# Autodesk Inventor assembly: leg_Left_femur_ass
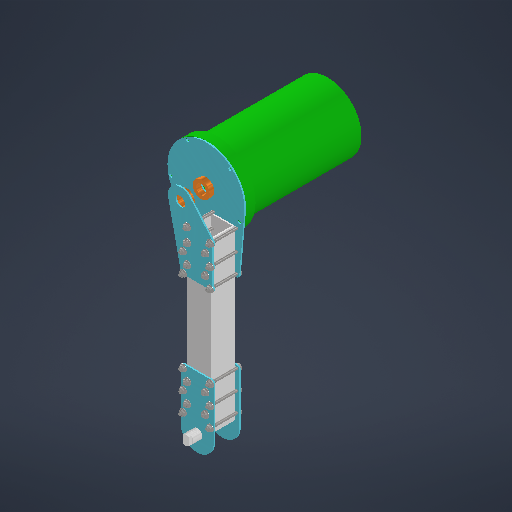
[picture p0: Inventor's stored thumbnail of the model, 512x512]
Saved by Autodesk Inventor 2026 (Build 300175000, 175)
## iProperties
Created: 2026-04-24
Part Number: leg_Left_femur_ass
Document SubType Name: Assembly
Designer: user
Mass: 5132.93 g
Surface Area: 5038.46 cm^2
Volume: 3187.52 cm^3
Density: 1.61032 g/cm^3
Author: user
## Documents named in this file (11)
- C:\Users\user\Documents\spider_metal\leg_femur\leg_Left_femur_ass.iam
- C:\Users\user\Documents\spider_metal\leg_femur\femur_profile.ipt
- C:\Users\user\Documents\spider_metal\leg_femur\femur_support_steel.ipt
- C:\Users\user\Documents\spider_metal\leg_femur\femur_motor_steel.ipt
- C:\Users\user\Documents\spider_metal\leg_femur\femur_outside_steel.ipt
- C:\Users\user\Documents\Inventor\Content Center Files\R2026\ru-RU\GOST 7805-70\Болт M6-6gx65 ГОСТ 7805-70.ipt
- C:\Users\user\Documents\Inventor\Content Center Files\R2026\ru-RU\Nut GOST R 50592-93\Гайка M6-6H ГОСТ Р 50592-93.ipt
- C:\Users\user\Documents\Inventor\Content Center Files\R2026\ru-RU\GOST 7798-70\Болт M6-6gx65 ГОСТ 7798-70.ipt
- C:\Users\user\Documents\spider_metal\leg_femur\shaft_femur.ipt
- C:\Users\user\Documents\spider_metal\body_parts\motor_mass.ipt
- C:\Users\user\Documents\spider_metal\body_parts\bearing_mass.ipt
## Components (49 placed, 10 different names)
1. femur_profile:1 — Жесткий:1, Жесткий:2, Жесткий:3, Жесткий:4, Совмещение:47, Совмещение:67
2. femur_support_steel:1 — Жесткий:1, Совмещение:22, Совмещение:24, Совмещение:26, Совмещение:28, Совмещение:30, Совмещение:32, Совмещение:34, Совмещение:36, Совмещение:38, Совмещение:40, С поворотом:3
3. femur_motor_steel:1 — Жесткий:4, Совмещение:1, Совмещение:2, Совмещение:3, Совмещение:4, Совмещение:5, Совмещение:6, Совмещение:7, Совмещение:8, Совмещение:9, Совмещение:10, Совмещение:11, Совмещение:12, Совмещение:13, Совмещение:14, Совмещение:15, Совмещение:16, Совмещение:17, Совмещение:18, Совмещение:19, Совмещение:20, Совмещение:21, Совмещение:23, Совмещение:25, Совмещение:27, Совмещение:29, Совмещение:31, Совмещение:33, Совмещение:35, Совмещение:37, Совмещение:39, С поворотом:1, Жесткий:6, С поворотом:2
4. femur_outside_steel:1 — Жесткий:2, Совмещение:62, Совмещение:64, Совмещение:66, Совмещение:68, Совмещение:70, Совмещение:72, Совмещение:74, Совмещение:76, Совмещение:78, Совмещение:80
5. femur_outside_steel:2 — Жесткий:3, Совмещение:41, Совмещение:42, Совмещение:43, Совмещение:44, Совмещение:45, Совмещение:46, Совмещение:48, Совмещение:49, Совмещение:50, Совмещение:51, Совмещение:52, Совмещение:53, Совмещение:54, Совмещение:55, Совмещение:56, Совмещение:57, Совмещение:58, Совмещение:59, Совмещение:60, Совмещение:61, Совмещение:63, Совмещение:65, Совмещение:69, Совмещение:71, Совмещение:73, Совмещение:75, Совмещение:77, Совмещение:79, Жесткий:5
6. shaft_femur:1 — Жесткий:5
7. motor_mass:1 — С поворотом:1, Жесткий:6
8. bearing_mass:1 — С поворотом:2
9. bearing_mass:2 — С поворотом:3
10. Болт ГОСТ 7798-70 - Отозвано M6-6gx65:1 — Совмещение:41, Совмещение:42
11. Гайка ГОСТ Р 50592-93 M6:11 — Совмещение:61, Совмещение:62
12. Болт ГОСТ 7798-70 - Отозвано M6-6gx65:2 — Совмещение:43, Совмещение:44
13. Болт ГОСТ 7798-70 - Отозвано M6-6gx65:3 — Совмещение:45, Совмещение:46
14. Болт ГОСТ 7798-70 - Отозвано M6-6gx65:4 — Совмещение:47, Совмещение:48
15. Болт ГОСТ 7798-70 - Отозвано M6-6gx65:5 — Совмещение:49, Совмещение:50
16. Болт ГОСТ 7798-70 - Отозвано M6-6gx65:6 — Совмещение:51, Совмещение:52
17. Болт ГОСТ 7798-70 - Отозвано M6-6gx65:7 — Совмещение:53, Совмещение:54
18. Болт ГОСТ 7798-70 - Отозвано M6-6gx65:8 — Совмещение:55, Совмещение:56
19. Болт ГОСТ 7798-70 - Отозвано M6-6gx65:9 — Совмещение:57, Совмещение:58
20. Болт ГОСТ 7798-70 - Отозвано M6-6gx65:10 — Совмещение:59, Совмещение:60
21. Гайка ГОСТ Р 50592-93 M6:12 — Совмещение:63, Совмещение:64
22. Гайка ГОСТ Р 50592-93 M6:13 — Совмещение:65, Совмещение:66
23. Гайка ГОСТ Р 50592-93 M6:14 — Совмещение:67, Совмещение:68
24. Гайка ГОСТ Р 50592-93 M6:15 — Совмещение:69, Совмещение:70
25. Гайка ГОСТ Р 50592-93 M6:16 — Совмещение:71, Совмещение:72
26. Гайка ГОСТ Р 50592-93 M6:17 — Совмещение:73, Совмещение:74
27. Гайка ГОСТ Р 50592-93 M6:18 — Совмещение:75, Совмещение:76
28. Гайка ГОСТ Р 50592-93 M6:19 — Совмещение:77, Совмещение:78
29. Гайка ГОСТ Р 50592-93 M6:20 — Совмещение:79, Совмещение:80
30. Болт ГОСТ 7805-70 M6-6gx65:1 — Совмещение:1, Совмещение:2
31. Гайка ГОСТ Р 50592-93 M6:1 — Совмещение:21, Совмещение:22
32. Болт ГОСТ 7805-70 M6-6gx65:2 — Совмещение:3, Совмещение:4
33. Болт ГОСТ 7805-70 M6-6gx65:3 — Совмещение:5, Совмещение:6
34. Болт ГОСТ 7805-70 M6-6gx65:4 — Совмещение:7, Совмещение:8
35. Болт ГОСТ 7805-70 M6-6gx65:5 — Совмещение:9, Совмещение:10
36. Болт ГОСТ 7805-70 M6-6gx65:6 — Совмещение:11, Совмещение:12
37. Болт ГОСТ 7805-70 M6-6gx65:7 — Совмещение:13, Совмещение:14
38. Болт ГОСТ 7805-70 M6-6gx65:8 — Совмещение:15, Совмещение:16
39. Болт ГОСТ 7805-70 M6-6gx65:9 — Совмещение:17, Совмещение:18
40. Болт ГОСТ 7805-70 M6-6gx65:10 — Совмещение:19, Совмещение:20
41. Гайка ГОСТ Р 50592-93 M6:2 — Совмещение:23, Совмещение:24
42. Гайка ГОСТ Р 50592-93 M6:3 — Совмещение:25, Совмещение:26
43. Гайка ГОСТ Р 50592-93 M6:4 — Совмещение:27, Совмещение:28
44. Гайка ГОСТ Р 50592-93 M6:5 — Совмещение:29, Совмещение:30
45. Гайка ГОСТ Р 50592-93 M6:6 — Совмещение:31, Совмещение:32
46. Гайка ГОСТ Р 50592-93 M6:7 — Совмещение:33, Совмещение:34
47. Гайка ГОСТ Р 50592-93 M6:8 — Совмещение:35, Совмещение:36
48. Гайка ГОСТ Р 50592-93 M6:9 — Совмещение:37, Совмещение:38
49. Гайка ГОСТ Р 50592-93 M6:10 — Совмещение:39, Совмещение:40
## Relationships (89: Mate 80, WeldJoint 6, RevoluteJoint 3)
- Жесткий:1 [WeldJoint]: femur_profile:1 ↔ femur_support_steel:1
- Жесткий:2 [WeldJoint]: femur_profile:1 ↔ femur_outside_steel:1
- Жесткий:3 [WeldJoint]: femur_profile:1 ↔ femur_outside_steel:2
- Жесткий:4 [WeldJoint]: femur_profile:1 ↔ femur_motor_steel:1
- Совмещение:1 [Mate]: femur_motor_steel:1 ↔ Болт ГОСТ 7805-70 M6-6gx65:1
- Совмещение:2 [Mate]: femur_motor_steel:1 ↔ Болт ГОСТ 7805-70 M6-6gx65:1
- Совмещение:3 [Mate]: femur_motor_steel:1 ↔ Болт ГОСТ 7805-70 M6-6gx65:2
- Совмещение:4 [Mate]: femur_motor_steel:1 ↔ Болт ГОСТ 7805-70 M6-6gx65:2
- Совмещение:5 [Mate]: femur_motor_steel:1 ↔ Болт ГОСТ 7805-70 M6-6gx65:3
- Совмещение:6 [Mate]: femur_motor_steel:1 ↔ Болт ГОСТ 7805-70 M6-6gx65:3
- Совмещение:7 [Mate]: femur_motor_steel:1 ↔ Болт ГОСТ 7805-70 M6-6gx65:4
- Совмещение:8 [Mate]: femur_motor_steel:1 ↔ Болт ГОСТ 7805-70 M6-6gx65:4
- Совмещение:9 [Mate]: femur_motor_steel:1 ↔ Болт ГОСТ 7805-70 M6-6gx65:5
- Совмещение:10 [Mate]: femur_motor_steel:1 ↔ Болт ГОСТ 7805-70 M6-6gx65:5
- Совмещение:11 [Mate]: femur_motor_steel:1 ↔ Болт ГОСТ 7805-70 M6-6gx65:6
- Совмещение:12 [Mate]: femur_motor_steel:1 ↔ Болт ГОСТ 7805-70 M6-6gx65:6
- Совмещение:13 [Mate]: femur_motor_steel:1 ↔ Болт ГОСТ 7805-70 M6-6gx65:7
- Совмещение:14 [Mate]: femur_motor_steel:1 ↔ Болт ГОСТ 7805-70 M6-6gx65:7
- Совмещение:15 [Mate]: femur_motor_steel:1 ↔ Болт ГОСТ 7805-70 M6-6gx65:8
- Совмещение:16 [Mate]: femur_motor_steel:1 ↔ Болт ГОСТ 7805-70 M6-6gx65:8
- Совмещение:17 [Mate]: femur_motor_steel:1 ↔ Болт ГОСТ 7805-70 M6-6gx65:9
- Совмещение:18 [Mate]: femur_motor_steel:1 ↔ Болт ГОСТ 7805-70 M6-6gx65:9
- Совмещение:19 [Mate]: femur_motor_steel:1 ↔ Болт ГОСТ 7805-70 M6-6gx65:10
- Совмещение:20 [Mate]: femur_motor_steel:1 ↔ Болт ГОСТ 7805-70 M6-6gx65:10
- Совмещение:21 [Mate]: femur_motor_steel:1 ↔ Гайка ГОСТ Р 50592-93 M6:1
- Совмещение:22 [Mate]: femur_support_steel:1 ↔ Гайка ГОСТ Р 50592-93 M6:1
- Совмещение:23 [Mate]: femur_motor_steel:1 ↔ Гайка ГОСТ Р 50592-93 M6:2
- Совмещение:24 [Mate]: femur_support_steel:1 ↔ Гайка ГОСТ Р 50592-93 M6:2
- Совмещение:25 [Mate]: femur_motor_steel:1 ↔ Гайка ГОСТ Р 50592-93 M6:3
- Совмещение:26 [Mate]: femur_support_steel:1 ↔ Гайка ГОСТ Р 50592-93 M6:3
- Совмещение:27 [Mate]: femur_motor_steel:1 ↔ Гайка ГОСТ Р 50592-93 M6:4
- Совмещение:28 [Mate]: femur_support_steel:1 ↔ Гайка ГОСТ Р 50592-93 M6:4
- Совмещение:29 [Mate]: femur_motor_steel:1 ↔ Гайка ГОСТ Р 50592-93 M6:5
- Совмещение:30 [Mate]: femur_support_steel:1 ↔ Гайка ГОСТ Р 50592-93 M6:5
- Совмещение:31 [Mate]: femur_motor_steel:1 ↔ Гайка ГОСТ Р 50592-93 M6:6
- Совмещение:32 [Mate]: femur_support_steel:1 ↔ Гайка ГОСТ Р 50592-93 M6:6
- Совмещение:33 [Mate]: femur_motor_steel:1 ↔ Гайка ГОСТ Р 50592-93 M6:7
- Совмещение:34 [Mate]: femur_support_steel:1 ↔ Гайка ГОСТ Р 50592-93 M6:7
- Совмещение:35 [Mate]: femur_motor_steel:1 ↔ Гайка ГОСТ Р 50592-93 M6:8
- Совмещение:36 [Mate]: femur_support_steel:1 ↔ Гайка ГОСТ Р 50592-93 M6:8
- Совмещение:37 [Mate]: femur_motor_steel:1 ↔ Гайка ГОСТ Р 50592-93 M6:9
- Совмещение:38 [Mate]: femur_support_steel:1 ↔ Гайка ГОСТ Р 50592-93 M6:9
- Совмещение:39 [Mate]: femur_motor_steel:1 ↔ Гайка ГОСТ Р 50592-93 M6:10
- Совмещение:40 [Mate]: femur_support_steel:1 ↔ Гайка ГОСТ Р 50592-93 M6:10
- Совмещение:41 [Mate]: femur_outside_steel:2 ↔ Болт ГОСТ 7798-70 - Отозвано M6-6gx65:1
- Совмещение:42 [Mate]: femur_outside_steel:2 ↔ Болт ГОСТ 7798-70 - Отозвано M6-6gx65:1
- Совмещение:43 [Mate]: femur_outside_steel:2 ↔ Болт ГОСТ 7798-70 - Отозвано M6-6gx65:2
- Совмещение:44 [Mate]: femur_outside_steel:2 ↔ Болт ГОСТ 7798-70 - Отозвано M6-6gx65:2
- Совмещение:45 [Mate]: femur_outside_steel:2 ↔ Болт ГОСТ 7798-70 - Отозвано M6-6gx65:3
- Совмещение:46 [Mate]: femur_outside_steel:2 ↔ Болт ГОСТ 7798-70 - Отозвано M6-6gx65:3
- Совмещение:47 [Mate]: femur_profile:1 ↔ Болт ГОСТ 7798-70 - Отозвано M6-6gx65:4
- Совмещение:48 [Mate]: femur_outside_steel:2 ↔ Болт ГОСТ 7798-70 - Отозвано M6-6gx65:4
- Совмещение:49 [Mate]: femur_outside_steel:2 ↔ Болт ГОСТ 7798-70 - Отозвано M6-6gx65:5
- Совмещение:50 [Mate]: femur_outside_steel:2 ↔ Болт ГОСТ 7798-70 - Отозвано M6-6gx65:5
- Совмещение:51 [Mate]: femur_outside_steel:2 ↔ Болт ГОСТ 7798-70 - Отозвано M6-6gx65:6
- Совмещение:52 [Mate]: femur_outside_steel:2 ↔ Болт ГОСТ 7798-70 - Отозвано M6-6gx65:6
- Совмещение:53 [Mate]: femur_outside_steel:2 ↔ Болт ГОСТ 7798-70 - Отозвано M6-6gx65:7
- Совмещение:54 [Mate]: femur_outside_steel:2 ↔ Болт ГОСТ 7798-70 - Отозвано M6-6gx65:7
- Совмещение:55 [Mate]: femur_outside_steel:2 ↔ Болт ГОСТ 7798-70 - Отозвано M6-6gx65:8
- Совмещение:56 [Mate]: femur_outside_steel:2 ↔ Болт ГОСТ 7798-70 - Отозвано M6-6gx65:8
- Совмещение:57 [Mate]: femur_outside_steel:2 ↔ Болт ГОСТ 7798-70 - Отозвано M6-6gx65:9
- Совмещение:58 [Mate]: femur_outside_steel:2 ↔ Болт ГОСТ 7798-70 - Отозвано M6-6gx65:9
- Совмещение:59 [Mate]: femur_outside_steel:2 ↔ Болт ГОСТ 7798-70 - Отозвано M6-6gx65:10
- Совмещение:60 [Mate]: femur_outside_steel:2 ↔ Болт ГОСТ 7798-70 - Отозвано M6-6gx65:10
- Совмещение:61 [Mate]: femur_outside_steel:2 ↔ Гайка ГОСТ Р 50592-93 M6:11
- Совмещение:62 [Mate]: femur_outside_steel:1 ↔ Гайка ГОСТ Р 50592-93 M6:11
- Совмещение:63 [Mate]: femur_outside_steel:2 ↔ Гайка ГОСТ Р 50592-93 M6:12
- Совмещение:64 [Mate]: femur_outside_steel:1 ↔ Гайка ГОСТ Р 50592-93 M6:12
- Совмещение:65 [Mate]: femur_outside_steel:2 ↔ Гайка ГОСТ Р 50592-93 M6:13
- Совмещение:66 [Mate]: femur_outside_steel:1 ↔ Гайка ГОСТ Р 50592-93 M6:13
- Совмещение:67 [Mate]: femur_profile:1 ↔ Гайка ГОСТ Р 50592-93 M6:14
- Совмещение:68 [Mate]: femur_outside_steel:1 ↔ Гайка ГОСТ Р 50592-93 M6:14
- Совмещение:69 [Mate]: femur_outside_steel:2 ↔ Гайка ГОСТ Р 50592-93 M6:15
- Совмещение:70 [Mate]: femur_outside_steel:1 ↔ Гайка ГОСТ Р 50592-93 M6:15
- Совмещение:71 [Mate]: femur_outside_steel:2 ↔ Гайка ГОСТ Р 50592-93 M6:16
- Совмещение:72 [Mate]: femur_outside_steel:1 ↔ Гайка ГОСТ Р 50592-93 M6:16
- Совмещение:73 [Mate]: femur_outside_steel:2 ↔ Гайка ГОСТ Р 50592-93 M6:17
- Совмещение:74 [Mate]: femur_outside_steel:1 ↔ Гайка ГОСТ Р 50592-93 M6:17
- Совмещение:75 [Mate]: femur_outside_steel:2 ↔ Гайка ГОСТ Р 50592-93 M6:18
- Совмещение:76 [Mate]: femur_outside_steel:1 ↔ Гайка ГОСТ Р 50592-93 M6:18
- Совмещение:77 [Mate]: femur_outside_steel:2 ↔ Гайка ГОСТ Р 50592-93 M6:19
- Совмещение:78 [Mate]: femur_outside_steel:1 ↔ Гайка ГОСТ Р 50592-93 M6:19
- Совмещение:79 [Mate]: femur_outside_steel:2 ↔ Гайка ГОСТ Р 50592-93 M6:20
- Совмещение:80 [Mate]: femur_outside_steel:1 ↔ Гайка ГОСТ Р 50592-93 M6:20
- Жесткий:5 [WeldJoint] (20 mm): femur_outside_steel:2 ↔ shaft_femur:1
- С поворотом:1 [RevoluteJoint]: femur_motor_steel:1 ↔ motor_mass:1
- Жесткий:6 [WeldJoint]: femur_motor_steel:1 ↔ motor_mass:1
- С поворотом:2 [RevoluteJoint]: femur_motor_steel:1 ↔ bearing_mass:1
- С поворотом:3 [RevoluteJoint]: femur_support_steel:1 ↔ bearing_mass:2
